# Autodesk Inventor assembly: motor assembly
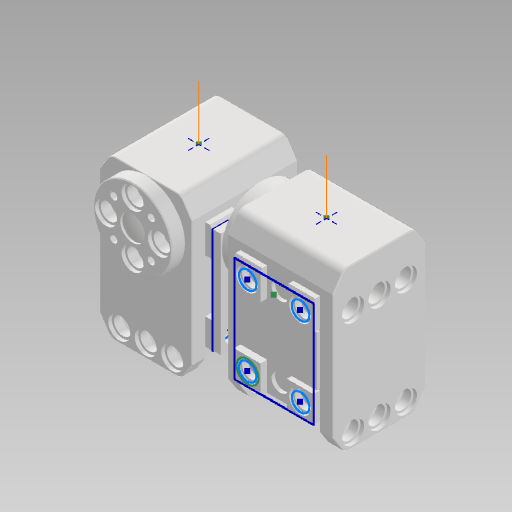
[picture p0: Inventor's stored thumbnail of the model, 512x512]
Saved by Autodesk Inventor 2021 (Build 250183000, 183)
## iProperties
Created: 2020-11-15
Part Number: motor assembly
Document SubType Name: Assembly
Designer: Paco
Mass: 33.2665 g
Surface Area: 117.108 cm^2
Volume: 33.2665 cm^3
Density: 1 g/cm^3
Author: Paco
## Documents named in this file (3)
- C:\Users\Kanenas\Desktop\IISRD_CAD_V\IISRD_V_v1\motor assembly.iam
- C:\Users\Kanenas\Desktop\IISRD_CAD_V\XL320XL-320.ipt
- C:\Users\Kanenas\Desktop\IISRD_CAD_V\IISRD_V_v1\XL_XL_interface.ipt
## Components (3 placed, 2 different names)
1. XL320XL-320:1 — Mate:1, Mate:2, Mate:3
2. XL_XL_interface:1 — Mate:1, Mate:2, Mate:3, Mate:4, Mate:5, Mate:6
3. XL320XL-320:2 — Mate:4, Mate:5, Mate:6
## Relationships (6: Mate 6)
- Mate:1: XL320XL-320:1 ↔ XL_XL_interface:1
- Mate:2: XL320XL-320:1 ↔ XL_XL_interface:1
- Mate:3: XL320XL-320:1 ↔ XL_XL_interface:1
- Mate:4: XL_XL_interface:1 ↔ XL320XL-320:2
- Mate:5: XL_XL_interface:1 ↔ XL320XL-320:2
- Mate:6: XL_XL_interface:1 ↔ XL320XL-320:2
